# Autodesk Inventor assembly: Assembly1
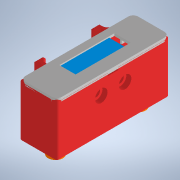
[picture p0: Inventor's stored thumbnail of the model, 180x180]
Saved by Autodesk Inventor 2020 (Build 240168000, 168)
## iProperties
Created: 2020-02-17
Part Number: Assembly1
Document SubType Name: Assembly
Designer: Timo
Author: Timo
## Documents named in this file (5)
- C:\Users\Timo\Documents\Inventor\IPT-Files\Electric\Assembly1.iam
- C:\Users\Timo\Documents\Inventor\IPT-Files\Electric\EndSwitchHousing_v02.ipt
- C:\Users\Timo\Documents\Inventor\IPT-Files\Electric\StereoBuchseEinbau.ipt
- C:\Users\Timo\Documents\Inventor\IPT-Files\Electric\EndSwitch_Model.ipt
- C:\Users\Timo\Documents\Inventor\IPT-Files\Electric\EndSwitchHousing_v02_TopPlate.ipt
## Components (5 placed, 4 different names)
1. EndSwitchHousing_v02:1 — Rotational:1, Rotational:2, Rotational:3, Rigid:1
2. StereoBuchseEinbau:1 — Rotational:2
3. StereoBuchseEinbau:2 — Rotational:1
4. EndSwitch_Model:1 — Rotational:3
5. EndSwitchHousing_v02_TopPlate:1 — Rigid:1
## Relationships (4: RevoluteJoint 3, WeldJoint 1)
- Rotational:1 [RevoluteJoint]: EndSwitchHousing_v02:1 ↔ StereoBuchseEinbau:2
- Rotational:2 [RevoluteJoint]: EndSwitchHousing_v02:1 ↔ StereoBuchseEinbau:1
- Rotational:3 [RevoluteJoint]: EndSwitchHousing_v02:1 ↔ EndSwitch_Model:1
- Rigid:1 [WeldJoint]: EndSwitchHousing_v02:1 ↔ EndSwitchHousing_v02_TopPlate:1
